# Autodesk Inventor assembly: ASY TZS 940 Filter column
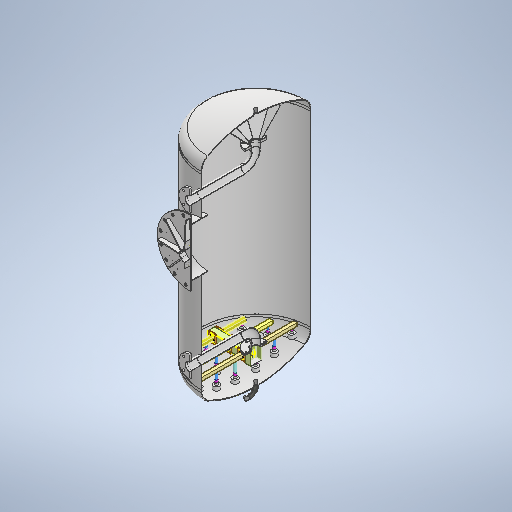
[picture p0: Inventor's stored thumbnail of the model, 512x512]
Saved by Autodesk Inventor 2025 (Build 290162010, 162A)
## iProperties
Created: 2025-02-13
Part Number: ASY TZS 940 Filter column
Document SubType Name: Assembly
Designer: pokla
Mass: 522904 g
Surface Area: 229381 cm^2
Volume: 66871 cm^3
Density: 7.81959 g/cm^3
Author: pokla
Revision Number: 2
## Documents named in this file (20)
- C:\Users\pokla\Documents\Inventor\TZS-Tazovskiy\Filter D940\ASY TZS 940 Filter column.iam
- C:\Users\pokla\Documents\Inventor\TZS-Tazovskiy\Filter D940\TZS 0903 accses hatch flange.ipt
- C:\Users\pokla\Documents\Inventor\TZS-Tazovskiy\Filter D940\TZS 0901 DIM Filter column.ipt
- C:\Users\pokla\Documents\Inventor\TZS-Tazovskiy\Filter D940\TZS 0904 accses hatch tube.ipt
- C:\Users\pokla\Documents\Inventor\TZS-Tazovskiy\Filter D940\TZS 0902 SHELL.ipt
- C:\Users\pokla\Documents\Inventor\TZS-Tazovskiy\Filter D940\TZS 0908 dished head.ipt
- C:\Users\pokla\Documents\Inventor\TZS-Tazovskiy\Filter D940\Fitting G1.ipt
- C:\Users\pokla\Documents\Inventor\TZS-Tazovskiy\Filter D940\TZS 0921 charging tube.ipt
- C:\Users\pokla\Documents\Inventor\TZS-Tazovskiy\Filter D940\ASY TZS 0980 Filter legs.iam
- C:\Users\pokla\Documents\Inventor\TZS-Tazovskiy\Filter D940\TZS 0922 charging flange round.ipt
- C:\Users\pokla\Documents\Inventor\TZS-Tazovskiy\Filter D940\sprinkler dummy.ipt
- C:\Users\pokla\Documents\Inventor\TZS-Tazovskiy\Filter D940\ASY TZS 0910 charging hatch.iam
- C:\Users\pokla\Documents\Inventor\TZS-Tazovskiy\Filter D940\TZS 0923 charging flange cup.ipt
- C:\Users\pokla\Documents\Inventor\TZS-Tazovskiy\Filter D940\TZS 0930 inner elbow.iam
- C:\Users\pokla\Documents\Inventor\TZS-Tazovskiy\Filter D940\ASY TZS 0940 FDS Top elbow.iam
- C:\Users\pokla\Documents\Inventor\TZS-Tazovskiy\Filter D940\TZS 0970 top funnel.iam
- C:\Users\pokla\Documents\Inventor\TZS-Tazovskiy\Filter D940\JIS B 2312 90 Deg Long Elbow Steel 32A x Sch 40.ipt
- C:\Users\pokla\Documents\Inventor\TZS-Tazovskiy\Filter D940\TZS 0991 accses hatch shell.ipt
- C:\Users\pokla\Documents\Inventor\TZS-Tazovskiy\Filter D940\FDS 940\ASY TZS 1650 filter-distribution-system 940.iam
- C:\Users\pokla\Documents\Inventor\TZS-Tazovskiy\Filter D940\Fitting G2.ipt
## Components (61 placed, 19 different names)
1. TZS 0901 DIM Filter column.ipt:1
2. TZS 0904 accses hatch tube.ipt:1 — Rigid:101, Rigid:106
3. TZS 0902 SHELL.ipt:1 — Flush:3, Flush:4, Rigid:99, Rigid:100, Rigid:101, Rigid:102, Rigid:103
4. TZS 0908 dished head.ipt:1 — Rigid:99, Mate:5, Rigid:105, Rotational:5
5. TZS 0908 dished head.ipt:2 — Rigid:100, Rigid:104
6. Fitting G1.ipt:1 — Rigid:104
7. TZS 0921 charging tube.ipt:1 — Rigid:32
8. TZS 0903 accses hatch flange.ipt:1 — Rotational:4, Rigid:106
9. ASY TZS 0980 Filter legs.iam:1 [sub-assembly] — Flush:2, Mate:4, Angle:1
10. TZS 0922 charging flange round.ipt:1 — Rigid:32, Rigid:51
11. ASY TZS 0910 charging hatch.iam:1 [sub-assembly] — Rotational:4
12. TZS 0923 charging flange cup.ipt:1 — Rigid:51
13. TZS 0930 inner elbow.iam:1 [sub-assembly] — Rigid:103, Rigid:108
14. ASY TZS 0940 FDS Top elbow.iam:1 [sub-assembly] — Rigid:102, Rigid:110
15. TZS 0970 top funnel.iam:1 [sub-assembly] — Rigid:110
16. JIS B 2312 90 Deg Long Elbow Steel 32A x Sch 40.ipt:1 — Rigid:105, Rigid:109
17. TZS 0991 accses hatch shell.ipt:1
18. ASY TZS 1650 filter-distribution-system 940.iam:1 [sub-assembly] — Rigid:108
19. Fitting G1.ipt:2 — Rotational:5
20. Fitting G2.ipt:1 — Rigid:109
21. sprinkler dummy.ipt:1
22. sprinkler dummy.ipt:2
23. sprinkler dummy.ipt:3
24. sprinkler dummy.ipt:4
25. sprinkler dummy.ipt:5
26. sprinkler dummy.ipt:6
27. sprinkler dummy.ipt:7
28. sprinkler dummy.ipt:8
29. sprinkler dummy.ipt:9
30. sprinkler dummy.ipt:10
31. sprinkler dummy.ipt:11
32. sprinkler dummy.ipt:12
33. sprinkler dummy.ipt:13
34. sprinkler dummy.ipt:14
35. sprinkler dummy.ipt:15
36. sprinkler dummy.ipt:16
37. sprinkler dummy.ipt:17
38. sprinkler dummy.ipt:18
39. sprinkler dummy.ipt:19
40. sprinkler dummy.ipt:20
41. sprinkler dummy.ipt:21
42. sprinkler dummy.ipt:22
43. sprinkler dummy.ipt:23
44. sprinkler dummy.ipt:24
45. sprinkler dummy.ipt:25
46. sprinkler dummy.ipt:26
47. sprinkler dummy.ipt:27
48. sprinkler dummy.ipt:28
49. sprinkler dummy.ipt:29
50. sprinkler dummy.ipt:30
51. sprinkler dummy.ipt:31
52. sprinkler dummy.ipt:32
53. sprinkler dummy.ipt:33
54. sprinkler dummy.ipt:34
55. sprinkler dummy.ipt:35
56. sprinkler dummy.ipt:36
57. sprinkler dummy.ipt:37
58. sprinkler dummy.ipt:38
59. sprinkler dummy.ipt:39
60. sprinkler dummy.ipt:40
61. sprinkler dummy.ipt:41
## Relationships (21: WeldJoint 13, Flush 3, Mate 2, RevoluteJoint 2, Angle 1)
- Flush:3: TZS 0902 SHELL.ipt:1
- Flush:4: TZS 0902 SHELL.ipt:1
- Flush:2: ASY TZS 0980 Filter legs.iam:1
- Rigid:32 [WeldJoint]: TZS 0921 charging tube.ipt:1 ↔ TZS 0922 charging flange round.ipt:1
- Mate:4: ASY TZS 0980 Filter legs.iam:1
- Angle:1 (145 deg): ASY TZS 0980 Filter legs.iam:1
- Rotational:4 [RevoluteJoint]: TZS 0903 accses hatch flange.ipt:1 ↔ ASY TZS 0910 charging hatch.iam:1
- Rigid:51 [WeldJoint]: TZS 0922 charging flange round.ipt:1 ↔ TZS 0923 charging flange cup.ipt:1
- Rigid:99 [WeldJoint]: TZS 0902 SHELL.ipt:1 ↔ TZS 0908 dished head.ipt:1
- Rigid:100 [WeldJoint]: TZS 0902 SHELL.ipt:1 ↔ TZS 0908 dished head.ipt:2
- Rigid:101 [WeldJoint]: TZS 0904 accses hatch tube.ipt:1 ↔ TZS 0902 SHELL.ipt:1
- Mate:5 (120 mm): TZS 0908 dished head.ipt:1
- Rigid:102 [WeldJoint] (98 mm): TZS 0902 SHELL.ipt:1 ↔ ASY TZS 0940 FDS Top elbow.iam:1
- Rigid:103 [WeldJoint] (98 mm): TZS 0902 SHELL.ipt:1 ↔ TZS 0930 inner elbow.iam:1
- Rigid:104 [WeldJoint]: TZS 0908 dished head.ipt:2 ↔ Fitting G1.ipt:1
- Rigid:105 [WeldJoint]: TZS 0908 dished head.ipt:1 ↔ JIS B 2312 90 Deg Long Elbow Steel 32A x Sch 40.ipt:1
- Rigid:106 [WeldJoint]: TZS 0904 accses hatch tube.ipt:1 ↔ TZS 0903 accses hatch flange.ipt:1
- Rigid:108 [WeldJoint]: TZS 0930 inner elbow.iam:1 ↔ ASY TZS 1650 filter-distribution-system 940.iam:1
- Rotational:5 [RevoluteJoint]: TZS 0908 dished head.ipt:1 ↔ Fitting G1.ipt:2
- Rigid:109 [WeldJoint]: JIS B 2312 90 Deg Long Elbow Steel 32A x Sch 40.ipt:1 ↔ Fitting G2.ipt:1
- Rigid:110 [WeldJoint]: ASY TZS 0940 FDS Top elbow.iam:1 ↔ TZS 0970 top funnel.iam:1
